# Autodesk Inventor assembly: Assembly
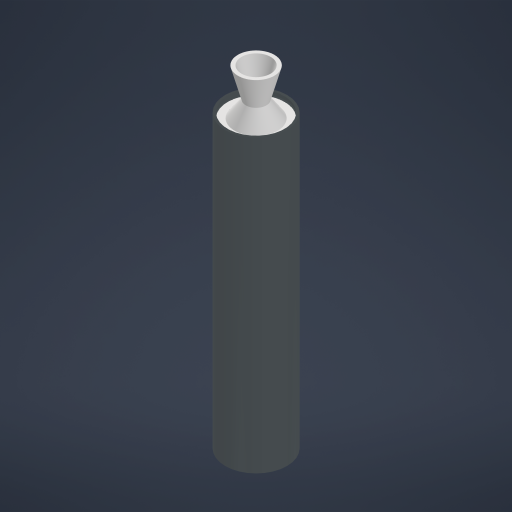
[picture p0: Inventor's stored thumbnail of the model, 512x512]
Saved by Autodesk Inventor 2023 (Build 270158000, 158)
## iProperties
Created: 2022-10-07
Part Number: Assembly
Document SubType Name: Assembly
Designer: washington
Author: washington
## Documents named in this file (4)
- C:\Users\washi\Documents\GitHub\airframeN2\CAD\Launch\Propulsion\Inventor files\Assembly.iam
- C:\Users\washi\Documents\GitHub\airframeN2\CAD\Launch\Propulsion\Inventor files\bulkhead.ipt
- C:\Users\washi\Documents\GitHub\airframeN2\CAD\Launch\Propulsion\Inventor files\casing.ipt
- C:\Users\washi\Documents\GitHub\airframeN2\CAD\Launch\Propulsion\Inventor files\nozzle.ipt
## Components (3 placed, 3 different names)
1. bulkhead:1 — Mate:3
2. casing:1 — Mate:1, Mate:2, Mate:3
3. nozzle:1 — Mate:1, Mate:2
## Relationships (3: Mate 3)
- Mate:1: casing:1 ↔ nozzle:1
- Mate:2: casing:1 ↔ nozzle:1
- Mate:3: bulkhead:1 ↔ casing:1
